# Autodesk Inventor assembly: LEG
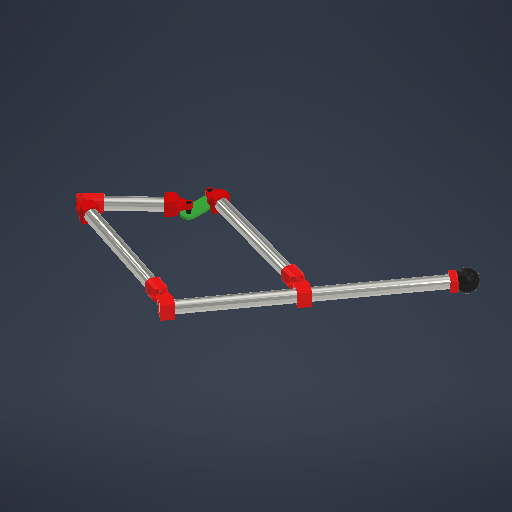
[picture p0: Inventor's stored thumbnail of the model, 512x512]
Saved by Autodesk Inventor 2027 (Build 310192060, 192F)
## iProperties
Created: 2026-08-01
Part Number: LEG
Document SubType Name: Assembly
Designer: User
Author: User
## Documents named in this file (9)
- G:\Github\Hot_dog\Hardware\Leg_concept\LEG.iam
- G:\Github\Hot_dog\Hardware\Leg_concept\Knee.ipt
- G:\Github\Hot_dog\Hardware\Leg_concept\foot.ipt
- G:\Github\Hot_dog\Hardware\Leg_concept\base.ipt
- G:\Github\Hot_dog\Hardware\Leg_concept\tibia.ipt
- G:\Github\Hot_dog\Hardware\Leg_concept\Connector_fill.ipt
- G:\Github\Hot_dog\Hardware\Leg_concept\Connector_hollow.ipt
- G:\Github\Hot_dog\Hardware\Leg_concept\short_tibia.ipt
- G:\Github\Hot_dog\Hardware\Leg_concept\connecting_rod.ipt
## Components (17 placed, 8 different names)
1. Connector_fill:1 — Sztywne:1, Obrotowe:4
2. Connector_hollow:1 — Sztywne:2, Obrotowe:8
3. tibia:1 — Sztywne:1, Sztywne:2
4. base:1 — Obrotowe:1, Obrotowe:2
5. Connector_fill:2 — Obrotowe:5
6. Connector_hollow:2 — Obrotowe:11
7. tibia:2
8. short_tibia:1 — Sztywne:5, Sztywne:6
9. Connector_fill:3 — Sztywne:6, Obrotowe:3
10. Connector_hollow:3 — Sztywne:5, Obrotowe:5
11. connecting_rod:1 — Obrotowe:1, Obrotowe:3
12. connecting_rod:2 — Obrotowe:2, Obrotowe:4
13. tibia:3 — Sztywne:7, Obrotowe:10
14. tibia:4 — Sztywne:7, Obrotowe:7, Obrotowe:9
15. Knee:1 — Obrotowe:7, Obrotowe:8
16. foot:1 — Obrotowe:9
17. Knee:2 — Obrotowe:10, Obrotowe:11
## Relationships (17: RevoluteJoint 10, WeldJoint 7)
- Sztywne:1 [WeldJoint]: Connector_fill:1 ↔ tibia:1
- Sztywne:2 [WeldJoint]: Connector_hollow:1 ↔ tibia:1
- [WeldJoint]: Connector_fill:2 ↔ tibia:2
- [WeldJoint]: Connector_hollow:2 ↔ tibia:2
- Sztywne:5 [WeldJoint]: short_tibia:1 ↔ Connector_hollow:3
- Sztywne:6 [WeldJoint]: short_tibia:1 ↔ Connector_fill:3
- Obrotowe:1 [RevoluteJoint]: base:1 ↔ connecting_rod:1
- Obrotowe:2 [RevoluteJoint]: base:1 ↔ connecting_rod:2
- Obrotowe:3 [RevoluteJoint]: Connector_fill:3 ↔ connecting_rod:1
- Obrotowe:4 [RevoluteJoint]: Connector_fill:1 ↔ connecting_rod:2
- Obrotowe:5 [RevoluteJoint]: Connector_fill:2 ↔ Connector_hollow:3
- Sztywne:7 [WeldJoint]: tibia:3 ↔ tibia:4
- Obrotowe:7 [RevoluteJoint] (8 mm): tibia:4 ↔ Knee:1
- Obrotowe:8 [RevoluteJoint]: Connector_hollow:1 ↔ Knee:1
- Obrotowe:9 [RevoluteJoint]: tibia:4 ↔ foot:1
- Obrotowe:10 [RevoluteJoint]: tibia:3 ↔ Knee:2
- Obrotowe:11 [RevoluteJoint]: Connector_hollow:2 ↔ Knee:2
## Named parameters: d36_d34 = 0 mm, d37_d35 = 0 mm
